# Autodesk Inventor assembly: A105EnsembleSupportLaser
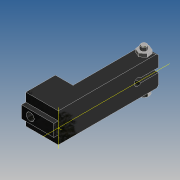
[picture p0: Inventor's stored thumbnail of the model, 180x180]
Saved by Autodesk Inventor 2017 (Build 210142000, 142)
## iProperties
Created: 2021-07-22
Part Number: A105EnsembleSupportLaser
Document SubType Name: Assembly
Designer: brice.dubuis
Author: brice.dubuis
## Documents named in this file (4)
- R:\Diploma\TD2021\SYND\brice.dubuis\Hardware\pièces mécaniques\FocalMeasure\A105EnsembleSupportLaser.iam
- R:\Diploma\TD2021\SYND\brice.dubuis\Hardware\pièces mécaniques\FocalMeasure\P116SupportFibre.ipt
- C:\Users\brice.dubuis\Documents\Inventor\ContentCenter\R2017\fr-FR\BS 4168(1)\BS 4168 - M4 x 25(1).ipt
- C:\Users\brice.dubuis\Documents\Inventor\ContentCenter\R2017\fr-FR\AS 1474(1)\AS 1474 - M4(1).ipt
## Components (3 placed, 3 different names)
1. P116SupportFibre:1 — Placage:1, Placage:2, Placage:4
2. BS 4168 : Pièce 1 Vis cylindrique à six pans creux - Métrique M4 x 25:1 — Placage:1, Placage:2, Placage:3
3. AS 1474 - Métrique M4:1 — Placage:3, Placage:4
## Relationships (4: Mate 4)
- Placage:1 [Mate]: P116SupportFibre:1 ↔ BS 4168 : Pièce 1 Vis cylindrique à six pans creux - Métrique M4 x 25:1
- Placage:2 [Mate]: P116SupportFibre:1 ↔ BS 4168 : Pièce 1 Vis cylindrique à six pans creux - Métrique M4 x 25:1
- Placage:3 [Mate]: BS 4168 : Pièce 1 Vis cylindrique à six pans creux - Métrique M4 x 25:1 ↔ AS 1474 - Métrique M4:1
- Placage:4 [Mate]: P116SupportFibre:1 ↔ AS 1474 - Métrique M4:1
